# Autodesk Inventor assembly: Mohinh3D
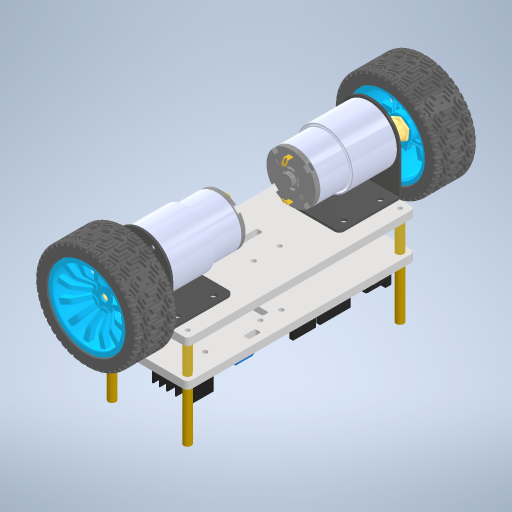
[picture p0: Inventor's stored thumbnail of the model, 512x512]
Saved by Autodesk Inventor 2023 (Build 270158000, 158)
## iProperties
Created: 2015-12-06
Part Number: Mohinh3D
Description: STEP AP214
Document SubType Name: Assembly
Designer: Admins
Sending System: SolidWorks 2014
Preprocessor: SwSTEP 2.0
Title: JGA25-371_ASM_(AP214).STEP
Revision Number: ANY
## Documents named in this file (10)
- D:\UNI\DoAn2\Mohinh3D.iam
- C:\Users\Admins\Downloads\65mm-wheel-1.snapshot.1\蓝色轮胎\65mm蓝色轮胎总装-实际外径68mm.ipt
- C:\Users\Admins\Downloads\l298-module-1.snapshot.14\L298N Stepper Motor Driver (Red).ipt
- C:\Users\Admins\Downloads\arduino-uno-r3-8.snapshot.2\Arduino Uno.ipt
- D:\UNI\DoAn2\DeDuoi.ipt
- D:\UNI\DoAn2\DeGiua.ipt
- C:\Users\Admins\Downloads\37-mm-dc-geared-motor-mounting-bracket-1.snapshot.11\37 mm DC Geared Motor Mounting Bracket.ipt
- C:\Users\Admins\Downloads\jgb37-520-1.snapshot.2\JGB37-520.ipt
- D:\UNI\DoAn2\Trudong30.ipt
- D:\UNI\DoAn2\Trudong35.ipt
## Components (18 placed, 9 different names)
1. 65mm蓝色轮胎总装-实际外径68mm:1 — Mate:29, Mate:30
2. 65mm蓝色轮胎总装-实际外径68mm:2 — Mate:28, Mate:31
3. L298N Stepper Motor Driver (Red):1 — Mate:42, Mate:43
4. Arduino Uno:1 — Mate:44, Mate:45
5. DeDuoi:1 — Mate:16, Mate:17, Mate:18, Mate:19, Mate:20, Mate:21, Mate:32, Mate:33, Mate:34, Mate:35, Mate:36, Mate:37, Mate:38, Mate:39
6. DeGiua:1 — Mate:40, Mate:41, Mate:42, Mate:43, Mate:44, Mate:45, Mate:46, Mate:47, Mate:48, Mate:49, Mate:51, Mate:52, Mate:53, Mate:54
7. 37 mm DC Geared Motor Mounting Bracket:1 — Mate:19, Mate:20, Mate:21, Mate:25, Mate:26, Mate:27
8. 37 mm DC Geared Motor Mounting Bracket:2 — Mate:16, Mate:17, Mate:18, Mate:22, Mate:23, Mate:24
9. JGB37-520:1 — Mate:25, Mate:26, Mate:27, Mate:29, Mate:30
10. JGB37-520:2 — Mate:22, Mate:23, Mate:24, Mate:28, Mate:31
11. Trudong30:1 — Mate:32, Mate:36
12. Trudong35:1 — Mate:49, Mate:52
13. Trudong30:2 — Mate:33, Mate:37, Mate:41
14. Trudong35:2 — Mate:48, Mate:53
15. Trudong30:3 — Mate:34, Mate:39, Mate:40, Mate:50
16. Trudong35:3 — Mate:47, Mate:54
17. Trudong30:4 — Mate:35, Mate:38
18. Trudong35:4 — Mate:46, Mate:50, Mate:51
## Relationships (39: Mate 39)
- Mate:16: DeDuoi:1 ↔ 37 mm DC Geared Motor Mounting Bracket:2
- Mate:17: DeDuoi:1 ↔ 37 mm DC Geared Motor Mounting Bracket:2
- Mate:18: DeDuoi:1 ↔ 37 mm DC Geared Motor Mounting Bracket:2
- Mate:19: DeDuoi:1 ↔ 37 mm DC Geared Motor Mounting Bracket:1
- Mate:20: DeDuoi:1 ↔ 37 mm DC Geared Motor Mounting Bracket:1
- Mate:21: DeDuoi:1 ↔ 37 mm DC Geared Motor Mounting Bracket:1
- Mate:22: 37 mm DC Geared Motor Mounting Bracket:2 ↔ JGB37-520:2
- Mate:23: 37 mm DC Geared Motor Mounting Bracket:2 ↔ JGB37-520:2
- Mate:24: 37 mm DC Geared Motor Mounting Bracket:2 ↔ JGB37-520:2
- Mate:25: 37 mm DC Geared Motor Mounting Bracket:1 ↔ JGB37-520:1
- Mate:26: 37 mm DC Geared Motor Mounting Bracket:1 ↔ JGB37-520:1
- Mate:27: 37 mm DC Geared Motor Mounting Bracket:1 ↔ JGB37-520:1
- Mate:28: 65mm蓝色轮胎总装-实际外径68mm:2 ↔ JGB37-520:2
- Mate:29: 65mm蓝色轮胎总装-实际外径68mm:1 ↔ JGB37-520:1
- Mate:30: 65mm蓝色轮胎总装-实际外径68mm:1 ↔ JGB37-520:1
- Mate:31: 65mm蓝色轮胎总装-实际外径68mm:2 ↔ JGB37-520:2
- Mate:32: DeDuoi:1 ↔ Trudong30:1
- Mate:33: DeDuoi:1 ↔ Trudong30:2
- Mate:34: DeDuoi:1 ↔ Trudong30:3
- Mate:35: DeDuoi:1 ↔ Trudong30:4
- Mate:36: DeDuoi:1 ↔ Trudong30:1
- Mate:37: DeDuoi:1 ↔ Trudong30:2
- Mate:38: DeDuoi:1 ↔ Trudong30:4
- Mate:39: DeDuoi:1 ↔ Trudong30:3
- Mate:40: DeGiua:1 ↔ Trudong30:3
- Mate:41: DeGiua:1 ↔ Trudong30:2
- Mate:42: L298N Stepper Motor Driver (Red):1 ↔ DeGiua:1
- Mate:43: L298N Stepper Motor Driver (Red):1 ↔ DeGiua:1
- Mate:44: Arduino Uno:1 ↔ DeGiua:1
- Mate:45: Arduino Uno:1 ↔ DeGiua:1
- Mate:46: DeGiua:1 ↔ Trudong35:4
- Mate:47: DeGiua:1 ↔ Trudong35:3
- Mate:48: DeGiua:1 ↔ Trudong35:2
- Mate:49: DeGiua:1 ↔ Trudong35:1
- Mate:50: Trudong30:3 ↔ Trudong35:4
- Mate:51: DeGiua:1 ↔ Trudong35:4
- Mate:52: DeGiua:1 ↔ Trudong35:1
- Mate:53: DeGiua:1 ↔ Trudong35:2
- Mate:54: DeGiua:1 ↔ Trudong35:3
